# Autodesk Inventor assembly: Caster
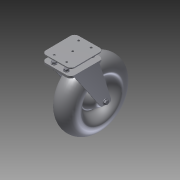
[picture p0: Inventor's stored thumbnail of the model, 180x180]
Saved by Autodesk Inventor 2012 (Build 160160000, 160)
## iProperties
Created: 2011-10-20
Part Number: Caster
Document SubType Name: Assembly
Designer: robotics
Author: robotics
## Documents named in this file (11)
- C:\Users\Ian Walters\Dropbox\CAD Inventor\Preseason Projects\Cart Competition Cart\Team 2374\Rotation Caster.iam
- C:\Users\Ian Walters\Dropbox\CAD Inventor\Preseason Projects\Cart Competition Cart\Team 2374\Wheel.ipt
- C:\Users\Ian Walters\Dropbox\CAD Inventor\Preseason Projects\Cart Competition Cart\Team 2374\Spacer - .5 x .25.ipt
- C:\Users\Ian Walters\Dropbox\CAD Inventor\Preseason Projects\Cart Competition Cart\Team 2374\Caster\Design Accelerator\Bolted Connection1.iam
- C:\Users\Ian Walters\Dropbox\CAD Inventor\Preseason Projects\Cart Competition Cart\Team 2374\Rotation Base.ipt
- C:\Users\Ian Walters\Dropbox\CAD Inventor\Preseason Projects\Cart Competition Cart\Team 2374\Rotation Top.ipt
- C:\Users\Ian Walters\Dropbox\CAD Inventor\Preseason Projects\Cart Competition Cart\Team 2374\Caster\Design Accelerator\Bolted Connection2.iam
- C:\Users\Ian Walters\Dropbox\CAD Inventor\Preseason Projects\Cart Competition Cart\Team 2374\Caster\Design Accelerator\Bolted Connection3.iam
- C:\Users\Ian Walters\Dropbox\CAD Inventor\Preseason Projects\Cart Competition Cart\Team 2374\Caster\Design Accelerator\Bolted Connection4.iam
- C:\Users\Ian Walters\Dropbox\CAD Inventor\Preseason Projects\Cart Competition Cart\Team 2374\Caster\Design Accelerator\Bolted Connection5.iam
- C:\Users\Ian Walters\Dropbox\CAD Inventor\Preseason Projects\Cart Competition Cart\Team 2374\Rotation Caster Flange.ipt
## Components (11 placed, 6 different names)
1. Rotation Caster Flange:1 — Mate:1, Mate:4, Mate:5, Mate:6, Mate:7, Flush:1, Mate:12, Flush:2, Mate:21, Mate:22
2. Wheel:1 — Mate:1, Mate:23
3. Spacer - .5 x .25:1 — Mate:4, Mate:5, Mate:23
4. Spacer - .5 x .25:2 — Mate:6, Mate:7
5. Bolted Connection:1 [sub-assembly] — Mate:21, Mate:22
6. Rotation Base:1 — Mate:10, Mate:11, Flush:1, Mate:12, Flush:2, Mate:24, Mate:25, Mate:26, Mate:27, Mate:28, Mate:29, Mate:30, Mate:31
7. Rotation Top:1 — Mate:10, Mate:11
8. Bolted Connection:2 [sub-assembly] — Mate:24, Mate:25
9. Bolted Connection:3 [sub-assembly] — Mate:26, Mate:27
10. Bolted Connection:4 [sub-assembly] — Mate:28, Mate:29
11. Bolted Connection:5 [sub-assembly] — Mate:30, Mate:31
## Relationships (21: Mate 19, Flush 2)
- Mate:1 (6.35 mm): Rotation Caster Flange:1 ↔ Wheel:1
- Mate:4: Rotation Caster Flange:1 ↔ Spacer - .5 x .25:1
- Mate:5: Rotation Caster Flange:1 ↔ Spacer - .5 x .25:1
- Mate:6: Rotation Caster Flange:1 ↔ Spacer - .5 x .25:2
- Mate:7: Rotation Caster Flange:1 ↔ Spacer - .5 x .25:2
- Mate:10: Rotation Base:1 ↔ Rotation Top:1
- Mate:11: Rotation Base:1 ↔ Rotation Top:1
- Flush:1: Rotation Caster Flange:1 ↔ Rotation Base:1
- Mate:12: Rotation Caster Flange:1 ↔ Rotation Base:1
- Flush:2: Rotation Caster Flange:1 ↔ Rotation Base:1
- Mate:21: Rotation Caster Flange:1 ↔ Bolted Connection:1
- Mate:22: Rotation Caster Flange:1 ↔ Bolted Connection:1
- Mate:23: Wheel:1 ↔ Spacer - .5 x .25:1
- Mate:24: Rotation Base:1 ↔ Bolted Connection:2
- Mate:25: Rotation Base:1 ↔ Bolted Connection:2
- Mate:26: Rotation Base:1 ↔ Bolted Connection:3
- Mate:27: Rotation Base:1 ↔ Bolted Connection:3
- Mate:28: Rotation Base:1 ↔ Bolted Connection:4
- Mate:29: Rotation Base:1 ↔ Bolted Connection:4
- Mate:30: Rotation Base:1 ↔ Bolted Connection:5
- Mate:31: Rotation Base:1 ↔ Bolted Connection:5
